# Autodesk Inventor assembly: robot
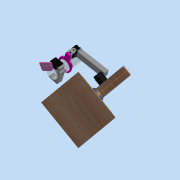
[picture p0: Inventor's stored thumbnail of the model, 180x180]
Saved by Autodesk Inventor 2017 (Build 210142000, 142)
## iProperties
Created: 2018-04-01
Part Number: robot
Document SubType Name: Assembly
Designer: franc
Author: franc
## Documents named in this file (15)
- C:\Users\Aegir\Documents\robotik 2017\git\2018\robot\robot.iam
- C:\Users\Aegir\Documents\robotik 2017\git\base_roulante\baseRoulante.iam
- C:\Users\Aegir\Documents\robotik 2017\git\2018\robot\socle-robot.ipt
- C:\Users\Aegir\Documents\robotik 2017\git\2018\robot\etage-bras.ipt
- C:\Users\Aegir\Documents\robotik 2017\git\2018\robot\traitement-eau\cylindre-stockage.ipt
- C:\Users\Aegir\Documents\robotik 2017\git\composants\AX12\AX12.iam
- C:\Users\Aegir\Documents\robotik 2017\git\2018\robot\traitement-eau\trappe.ipt
- C:\Users\Aegir\Documents\robotik 2017\git\composants\AX12\F3.ipt
- C:\Users\Aegir\Documents\robotik 2017\git\2018\robot\traitement-eau\support-trappe.ipt
- C:\Users\Aegir\Documents\robotik 2017\git\composants\AX12\F2.ipt
- C:\Users\Aegir\Documents\robotik 2017\git\composants\AX12\ax12_wheel.ipt
- C:\Users\Aegir\Documents\robotik 2017\git\composants\AX12\ax12_box.ipt
- C:\Users\Aegir\Documents\robotik 2017\git\2018\robot\traitement-eau\rotation-recuperation.ipt
- C:\Users\Aegir\Documents\robotik 2017\git\2018\robot\traitement-eau\bras.ipt
- C:\Users\Aegir\Documents\robotik 2017\git\2018\robot\traitement-eau\fixation-bras.ipt
## Components (15 placed, 14 different names)
1. baseRoulante:1 [sub-assembly] — Affleurement:1, Affleurement:2, Placage:1, Angle:1
2. socle-robot:1 — Affleurement:1, Affleurement:2, Placage:1, Affleurement:3, Placage:21, Placage:22
3. etage-bras:1 — Affleurement:3, Angle:1, Placage:20, Affleurement:10, Placage:21, Placage:22, Affleurement:11
4. cylindre-stockage:1
5. AX12:1 [sub-assembly]
6. trappe:1
7. F3:1
8. support-trappe:1
9. F2:1
10. ax12_wheel:1
11. ax12_box:1
12. rotation-recuperation:1
13. bras:1 — Placage:23
14. AX12:2 [sub-assembly] — Placage:23
15. fixation-bras:1 — Placage:20, Affleurement:10, Affleurement:11
## Relationships (41: Mate 23, Flush 10, Tangent 6, Angle 1, Insert 1)
- Affleurement:1 [Flush] (5 mm): baseRoulante:1 ↔ socle-robot:1
- Affleurement:2 [Flush] (54 mm): baseRoulante:1 ↔ socle-robot:1
- Placage:1 [Mate]: baseRoulante:1 ↔ socle-robot:1
- Affleurement:3 [Flush] (5 mm): socle-robot:1 ↔ etage-bras:1
- Angle:1 (0 deg): baseRoulante:1 ↔ etage-bras:1
- [Flush]: cylindre-stockage:1 ↔ AX12:1
- [Tangent]: AX12:1 ↔ trappe:1
- [Tangent]: AX12:1 ↔ trappe:1
- [Mate]: AX12:1 ↔ trappe:1
- [Mate]: AX12:1 ↔ F3:1
- [Mate]: AX12:1 ↔ F3:1
- [Mate]: AX12:1 ↔ F3:1
- [Tangent] (1 mm): cylindre-stockage:1 ↔ AX12:1
- [Tangent]: cylindre-stockage:1 ↔ AX12:1
- [Mate]: F3:1 ↔ support-trappe:1
- [Flush]: F3:1 ↔ support-trappe:1
- [Mate]: F3:1 ↔ support-trappe:1
- [Insert]: ax12_wheel:1 ↔ ax12_box:1
- [Mate]: F2:1 ↔ ax12_wheel:1
- [Mate]: F2:1 ↔ ax12_wheel:1
- [Mate]: F2:1 ↔ ax12_wheel:1
- [Tangent] (1 mm): cylindre-stockage:1 ↔ F2:1
- [Flush] (87.5 mm): cylindre-stockage:1 ↔ F2:1
- [Flush] (25.5 mm): support-trappe:1 ↔ F2:1
- [Mate]: F2:1 ↔ rotation-recuperation:1
- [Flush]: F2:1 ↔ rotation-recuperation:1
- [Mate]: ax12_box:1 ↔ bras:1
- [Mate]: ax12_box:1 ↔ bras:1
- [Mate]: ax12_box:1 ↔ bras:1
- [Mate]: bras:1 ↔ AX12:2
- [Tangent] (6 mm): bras:1 ↔ AX12:2
- [Mate]: AX12:2 ↔ fixation-bras:1
- [Mate]: AX12:2 ↔ fixation-bras:1
- [Mate]: AX12:2 ↔ fixation-bras:1
- [Mate]: cylindre-stockage:1 ↔ rotation-recuperation:1
- Placage:20 [Mate]: etage-bras:1 ↔ fixation-bras:1
- Affleurement:10 [Flush]: etage-bras:1 ↔ fixation-bras:1
- Placage:21 [Mate] (200 mm): socle-robot:1 ↔ etage-bras:1
- Placage:22 [Mate]: socle-robot:1 ↔ etage-bras:1
- Affleurement:11 [Flush] (60 mm): etage-bras:1 ↔ fixation-bras:1
- Placage:23 [Mate]: bras:1 ↔ AX12:2
## Named parameters: d89_d23 = 0 mm, d90_d24 = 0 mm, d28_d1 = 0 mm
